# Autodesk Inventor assembly: 00_ESP3-CAM
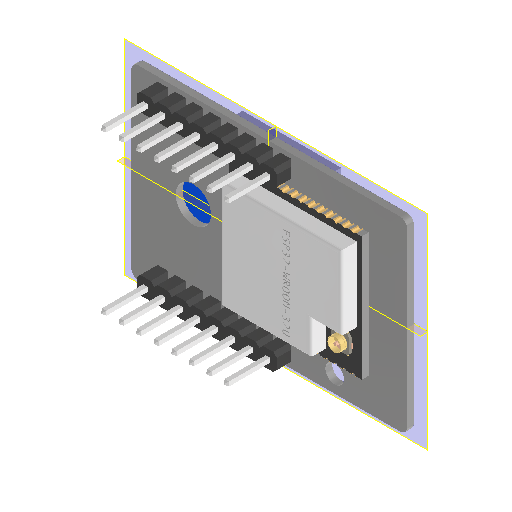
[picture p0: Inventor's stored thumbnail of the model, 512x512]
Saved by Autodesk Inventor 2022 (Build 260153000, 153)
## iProperties
Created: 2019-05-06
Part Number: 00_ESP3-CAM
Document SubType Name: Assembly
Designer: diederichbenedict
Sending System: Autodesk Translation Framework v8.2.0.1029
Preprocessor: ST-DEVELOPER v18
Title: /Users/janjezek/Downloads/ESP3-CAM v4.step
Author: jezekjan
## Documents named in this file (7)
- C:\Users\UC2\Documents\GitHub\Matchboxscope\INVENTOR\00_ESP3-CAM.iam
- C:\Users\UC2\Documents\GitHub\Matchboxscope\INVENTOR\Pin Header 4 x 1 TH 2.54mm Pitch v1.ipt
- C:\Users\UC2\Documents\GitHub\Matchboxscope\INVENTOR\ESp32-WROOM-32U v3 v1.iam
- C:\Users\UC2\Documents\GitHub\Matchboxscope\INVENTOR\MicroSD Slot v1.iam
- C:\Users\UC2\Documents\GitHub\Matchboxscope\INVENTOR\Micro SD-Card v1.ipt
- C:\Users\UC2\Documents\GitHub\Matchboxscope\INVENTOR\Bauteil50.ipt
- C:\Users\UC2\Documents\GitHub\Matchboxscope\INVENTOR\Anglerfish_Cameraspacer.ipt
## Components (9 placed, 6 different names)
1. Pin Header 4 x 1 TH 2.54mm Pitch v1:1
2. Pin Header 4 x 1 TH 2.54mm Pitch v1:2
3. Pin Header 4 x 1 TH 2.54mm Pitch v1:3
4. Pin Header 4 x 1 TH 2.54mm Pitch v1:4
5. ESp32-WROOM-32U v3 v1:1 [sub-assembly]
6. MicroSD Slot v1:1 [sub-assembly]
7. Micro SD-Card v1:1
8. Bauteil50 — Fluchtend:1, Fluchtend:2
9. Anglerfish_Cameraspacer:1 — Fluchtend:1, Fluchtend:2
## Relationships (2: Flush 2)
- Fluchtend:1 [Flush]: Bauteil50 ↔ Anglerfish_Cameraspacer:1
- Fluchtend:2 [Flush]: Bauteil50 ↔ Anglerfish_Cameraspacer:1
